# Autodesk Inventor assembly: Lift.01.00.00.00
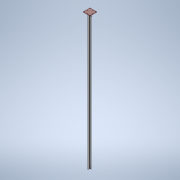
[picture p0: Inventor's stored thumbnail of the model, 180x180]
Saved by Autodesk Inventor 2021 (Build 250183000, 183)
## iProperties
Created: 2020-09-20
Part Number: Lift.01.00.00.00
Document SubType Name: Assembly
Designer: Kostya
Author: Kostya
## Documents named in this file (3)
- C:\Lift\Lift.01.00.00.00.iam
- C:\Lift\Lift.01.00.00.01.ipt
- C:\Lift\Lift.01.00.00.00.ipt
## Components (2 placed, 2 different names)
1. Lift.01.00.00.01:1 — Совмещение:1, Совмещение:2, Совмещение:3, Заподлицо:1, Совмещение:4
2. Lift.01.00.00.00:1 — Совмещение:3, Заподлицо:1, Совмещение:4
## Relationships (5: Mate 4, Flush 1)
- Совмещение:1 [Mate]: Lift.01.00.00.01:1
- Совмещение:2 [Mate]: Lift.01.00.00.01:1
- Совмещение:3 [Mate]: Lift.01.00.00.01:1 ↔ Lift.01.00.00.00:1
- Заподлицо:1 [Flush]: Lift.01.00.00.01:1 ↔ Lift.01.00.00.00:1
- Совмещение:4 [Mate]: Lift.01.00.00.01:1 ↔ Lift.01.00.00.00:1
